# Autodesk Inventor assembly: Filament Lift Extruder
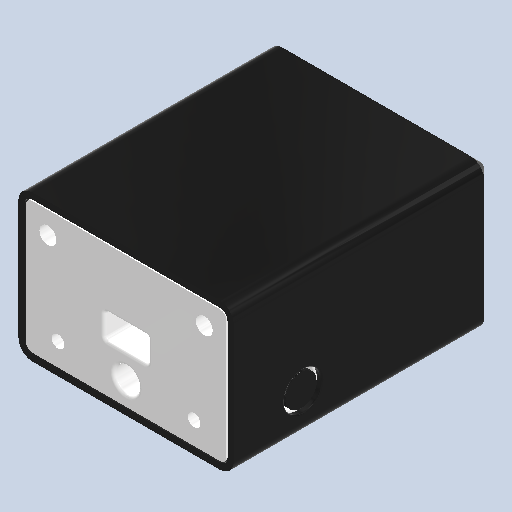
[picture p0: Inventor's stored thumbnail of the model, 512x512]
Saved by Autodesk Inventor 2024 (Build 280153000, 153)
## iProperties
Created: 2025-01-02
Part Number: Filament Lift Extruder
Document SubType Name: Assembly
Designer: Ishaan
Author: Ishaan
## Documents named in this file (5)
- E:\Projects\Axiom--IDEX-3D-Printer\CAD\06 - Filament Path\Filament Lift Extruder.iam
- E:\Projects\Axiom--IDEX-3D-Printer\CAD\00 - COTS Components\HGXLite Extruder\HGX-extruder\HGX-extruder.ipt
- E:\Projects\Axiom--IDEX-3D-Printer\CAD\00 - COTS Components\Microswitch\MS085xx02FxxxS1A.ipt
- E:\Projects\Axiom--IDEX-3D-Printer\CAD\06 - Filament Path\Lift Extruder Filament Guide.ipt
- E:\Projects\Axiom--IDEX-3D-Printer\CAD\00 - COTS Components\5p5mm Ball Bearing\5p5mm Ball Bearing.ipt
## Components (4 placed, 4 different names)
1. HGX-extruder:1 — Insert:1, Insert:2
2. MS085xx02FxxxS1A:1 — Insert:3, Insert:4
3. Lift Extruder Filament Guide:1 — Insert:1, Insert:2, Insert:3, Insert:4, Mate:1
4. 5p5mm Ball Bearing:1 — Mate:1
## Relationships (5: Insert 4, Mate 1)
- Insert:1: HGX-extruder:1 ↔ Lift Extruder Filament Guide:1
- Insert:2: HGX-extruder:1 ↔ Lift Extruder Filament Guide:1
- Insert:3: MS085xx02FxxxS1A:1 ↔ Lift Extruder Filament Guide:1
- Insert:4: MS085xx02FxxxS1A:1 ↔ Lift Extruder Filament Guide:1
- Mate:1: Lift Extruder Filament Guide:1 ↔ 5p5mm Ball Bearing:1
